# Autodesk Inventor assembly: Sensor_PCB
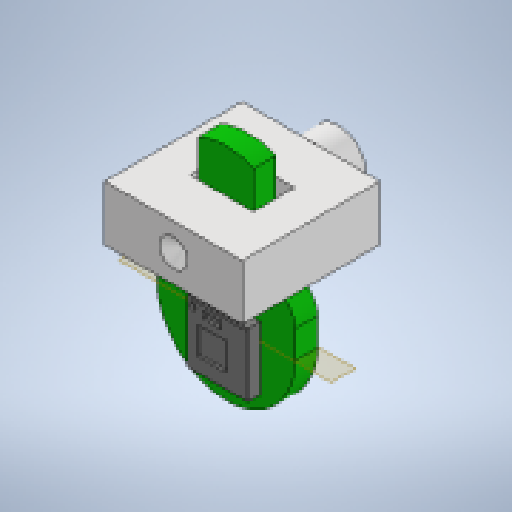
[picture p0: Inventor's stored thumbnail of the model, 512x512]
Saved by Autodesk Inventor 2024 (Build 280153000, 153)
## iProperties
Created: 2025-02-15
Part Number: Sensor_PCB
Document SubType Name: Assembly
Designer: XxPan
Author: XxPan
## Documents named in this file (5)
- C:\Users\XxPan\OneDrive - McMaster University\4OI6\InkSync\case\Sensor_PCB.iam
- C:\Users\XxPan\OneDrive - McMaster University\4OI6\InkSync\case\Force_sensor.ipt
- C:\Users\XxPan\OneDrive - McMaster University\4OI6\InkSync\case\Optical_sensor.ipt
- C:\Users\XxPan\OneDrive - McMaster University\4OI6\InkSync\case\Sensor_PCB.ipt
- C:\Users\XxPan\OneDrive - McMaster University\4OI6\InkSync\case\Pen_nib_stopper.ipt
## Components (4 placed, 4 different names)
1. Force_sensor:1 — Mate:2, Flush:2, Flush:3
2. Optical_sensor:1 — Mate:1, Flush:1, Flush:4
3. Sensor_PCB:1 — Mate:1, Mate:2, Flush:1, Flush:2, Flush:3, Mate:3, Angle:1, Mate:4, Mate:5
4. Pen_nib_stopper:1 — Mate:4, Mate:5
## Relationships (10: Mate 5, Flush 4, Angle 1)
- Mate:1: Optical_sensor:1 ↔ Sensor_PCB:1
- Mate:2: Force_sensor:1 ↔ Sensor_PCB:1
- Flush:1: Optical_sensor:1 ↔ Sensor_PCB:1
- Flush:2: Force_sensor:1 ↔ Sensor_PCB:1
- Flush:3: Force_sensor:1 ↔ Sensor_PCB:1
- Mate:3: Sensor_PCB:1
- Angle:1 (0 deg): Sensor_PCB:1
- Flush:4: Optical_sensor:1
- Mate:4: Sensor_PCB:1 ↔ Pen_nib_stopper:1
- Mate:5 (0.2 mm): Sensor_PCB:1 ↔ Pen_nib_stopper:1
